# Autodesk Inventor assembly: OBG-Dribbler und Chipper v2
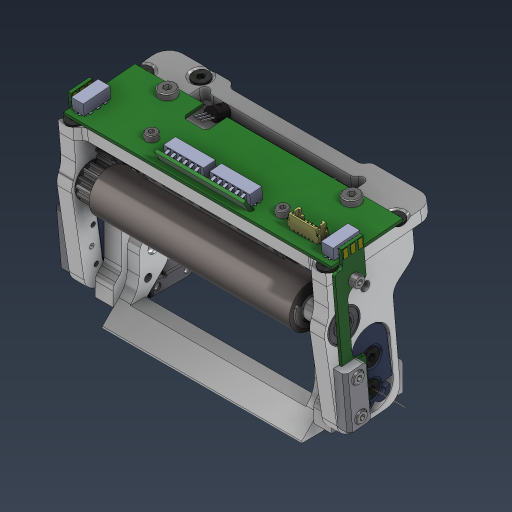
[picture p0: Inventor's stored thumbnail of the model, 512x512]
Saved by Autodesk Inventor 2023.1 (Build 271208000, 208)
## iProperties
Part Number: OBG-Dribbler und Chipper v2
Material: Generisch
Document SubType Name: Assembly
Designer: rYan
Mass: 268.659 g
Surface Area: 545.327 cm^2
Volume: 68.049 cm^3
Author: rYan
## Documents named in this file (3)
- D:\TIGERsGIT\Hardware\mechanik\2020\Inventor\Robot\Dribbler\OBG-Dribbler und Chipper v2.iam
- D:\TIGERsGIT\Hardware\mechanik\2020\Inventor\Robot\Dribbler\UBG-Dribblerhalter v2.iam
- D:\TIGERsGIT\Hardware\mechanik\2020\Inventor\Robot\Dribbler\UBG-Dribbler v2.iam
## Components (2 placed, 2 different names)
1. UBG-Dribbler v2:1 [sub-assembly] — Passend:1, Passend:5, Winkel:1
2. UBG-Dribblerhalter v2:1 [sub-assembly] — Passend:3, Fluchtend:1, Passend:4, Passend:5, Winkel:1
## Relationships (6: Mate 4, Flush 1, Angle 1)
- Passend:1 [Mate]: UBG-Dribbler v2:1
- Passend:3 [Mate]: UBG-Dribblerhalter v2:1
- Fluchtend:1 [Flush]: UBG-Dribblerhalter v2:1
- Passend:4 [Mate]: UBG-Dribblerhalter v2:1
- Passend:5 [Mate]: UBG-Dribbler v2:1 ↔ UBG-Dribblerhalter v2:1
- Winkel:1 [Angle] (-5 deg): UBG-Dribbler v2:1 ↔ UBG-Dribblerhalter v2:1
